# Autodesk Inventor assembly: Motor-GM15BY
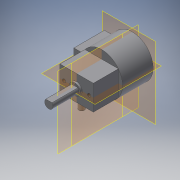
[picture p0: Inventor's stored thumbnail of the model, 180x180]
Saved by Autodesk Inventor 2019 (Build 230136000, 136)
## iProperties
Created: 2021-01-03
Part Number: Motor-GM15BY
Document SubType Name: Assembly
Designer: Sam
Author: Sam
## Documents named in this file (3)
- D:\OneDrive\MSc Robotics\GIC\RobotKinematics-Remote\3D CAD\Motor-GM15BY.iam
- D:\OneDrive\MSc Robotics\GIC\RobotKinematics-Remote\3D CAD\Motor-Body.ipt
- D:\OneDrive\MSc Robotics\GIC\RobotKinematics-Remote\3D CAD\Motor-Shaft.ipt
## Components (2 placed, 2 different names)
1. Motor-Body:1 — Flush:1, Flush:2, Rotational:1
2. Motor-Shaft:1 — Flush:1, Flush:2, Rotational:1
## Relationships (3: Flush 2, RevoluteJoint 1)
- Flush:1: Motor-Body:1 ↔ Motor-Shaft:1
- Flush:2: Motor-Body:1 ↔ Motor-Shaft:1
- Rotational:1 [RevoluteJoint] (-9.3 mm): Motor-Body:1 ↔ Motor-Shaft:1
